# Autodesk Inventor assembly: gripperReference
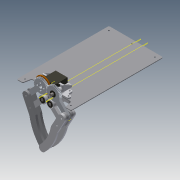
[picture p0: Inventor's stored thumbnail of the model, 180x180]
Saved by Autodesk Inventor 2018 (Build 220112000, 112)
## iProperties
Created: 2020-01-19
Part Number: gripperReference
Document SubType Name: Assembly
Designer: anirudh
Author: anirudh
## Documents named in this file (15)
- D:\Silicon Sharks\2019-2020\Gripper\gripperReference.iam
- D:\Silicon Sharks\2019-2020\Gripper\gripperServo.ipt
- D:\Silicon Sharks\2019-2020\Gripper\REV-41-1363.ipt
- D:\Silicon Sharks\2019-2020\Gripper\gripperPart1.ipt
- D:\Silicon Sharks\2019-2020\prototype3\bottomMountingPlate.ipt
- D:\Silicon Sharks\2019-2020\Gripper\gripperPart2.ipt
- D:\Silicon Sharks\2019-2020\Gripper\am-3377 6x12x4 Flanged Bearing.ipt
- D:\Silicon Sharks\2019-2020\Gripper\gripperPart3.ipt
- D:\Silicon Sharks\2019-2020\Gripper\gripperPart4.ipt
- D:\Silicon Sharks\2019-2020\Gripper\6mm-1inAxle.ipt
- D:\Silicon Sharks\2019-2020\Gripper\gripperPart5.ipt
- D:\Silicon Sharks\2019-2020\Gripper\spacer.ipt
- D:\Silicon Sharks\2019-2020\Gripper\servoMount.ipt
- D:\Silicon Sharks\2019-2020\Gripper\servoMount2.ipt
- D:\Silicon Sharks\2019-2020\Gripper\axleMount.ipt
## Components (26 placed, 14 different names)
1. gripperServo:1 — Mate:1, Mate:2, Mate:6, Flush:1, Flush:4, Mate:62, Mate:63, Mate:65, Mate:66
2. REV-41-1363:1 — Mate:1, Mate:2, Mate:3, Mate:4, Mate:5
3. gripperPart1:1 — Mate:3, Mate:4, Mate:5, Flush:7, Mate:18, Flush:10, Mate:34, Mate:35, Mate:38
4. bottomMountingPlate:1 — Mate:6, Flush:1, Flush:4, Flush:6, Mate:11, Flush:8, Mate:20, Mate:21, Flush:9, Mate:61, Mate:64, Flush:14
5. gripperPart2:1 — Flush:7, Mate:11, Mate:13, Mate:14, Mate:15, Mate:16, Mate:17, Mate:19, Flush:11, Mate:56, Mate:58, Mate:60
6. am-3377 6x12x4 Flanged Bearing:1 — Mate:14, Mate:15, Mate:68
7. am-3377 6x12x4 Flanged Bearing:2 — Mate:16, Mate:17, Mate:67
8. gripperPart3:1 — Mate:20, Mate:21, Flush:9, Mate:22, Mate:31, Flush:12, Mate:32, Flush:13, Mate:33
9. gripperPart4:1 — Flush:10, Mate:22, Mate:23, Mate:24, Mate:25, Mate:26, Mate:36, Mate:37, Mate:39
10. gripperPart4:2 — Mate:27, Mate:28, Mate:29, Mate:30, Flush:11, Mate:40, Mate:41, Mate:46, Mate:47
11. am-3377 6x12x4 Flanged Bearing:3 — Mate:25, Mate:26
12. am-3377 6x12x4 Flanged Bearing:4 — Mate:29, Mate:30, Mate:31
13. am-3377 6x12x4 Flanged Bearing:5 — Mate:27, Mate:28
14. am-3377 6x12x4 Flanged Bearing:6 — Mate:23, Mate:24
15. 6mm-1inAxle:1 — Flush:13, Mate:33
16. 6mm-1inAxle:2 — Flush:12, Mate:32
17. gripperPart5:1 — Mate:34, Mate:35, Mate:36
18. gripperPart5:2 — Mate:37, Mate:38, Mate:39
19. spacer:1 — Mate:40, Mate:41, Mate:50, Mate:54, Mate:55, Mate:60
20. spacer:4 — Mate:46, Mate:47, Mate:53, Mate:57, Mate:59
21. gripperPart5:3 — Mate:53, Mate:57, Mate:58, Mate:59
22. gripperPart5:4 — Mate:50, Mate:54, Mate:55, Mate:56
23. servoMount:1 — Mate:61, Mate:62, Mate:63
24. servoMount2:1 — Mate:64, Mate:65, Mate:66
25. axleMount:1 — Mate:67, Flush:14, Flush:15
26. 6mm-1inAxle:3 — Flush:15, Mate:68
## Relationships (67: Mate 55, Flush 12)
- Mate:1: gripperServo:1 ↔ REV-41-1363:1
- Mate:2: gripperServo:1 ↔ REV-41-1363:1
- Mate:3: REV-41-1363:1 ↔ gripperPart1:1
- Mate:4: REV-41-1363:1 ↔ gripperPart1:1
- Mate:5: REV-41-1363:1 ↔ gripperPart1:1
- Mate:6: gripperServo:1 ↔ bottomMountingPlate:1
- Flush:1: gripperServo:1 ↔ bottomMountingPlate:1
- Flush:4: gripperServo:1 ↔ bottomMountingPlate:1
- Flush:6 (7.493 mm): bottomMountingPlate:1
- Flush:7: gripperPart1:1 ↔ gripperPart2:1
- Mate:11: bottomMountingPlate:1 ↔ gripperPart2:1
- Mate:13: gripperPart2:1
- Mate:14: gripperPart2:1 ↔ am-3377 6x12x4 Flanged Bearing:1
- Mate:15: gripperPart2:1 ↔ am-3377 6x12x4 Flanged Bearing:1
- Mate:16: gripperPart2:1 ↔ am-3377 6x12x4 Flanged Bearing:2
- Mate:17: gripperPart2:1 ↔ am-3377 6x12x4 Flanged Bearing:2
- Flush:8 (23.241 mm): bottomMountingPlate:1
- Mate:18: gripperPart1:1
- Mate:19: gripperPart2:1
- Mate:20: bottomMountingPlate:1 ↔ gripperPart3:1
- Mate:21: bottomMountingPlate:1 ↔ gripperPart3:1
- Flush:9: bottomMountingPlate:1 ↔ gripperPart3:1
- Flush:10: gripperPart1:1 ↔ gripperPart4:1
- Mate:22: gripperPart3:1 ↔ gripperPart4:1
- Mate:23: gripperPart4:1 ↔ am-3377 6x12x4 Flanged Bearing:6
- Mate:24: gripperPart4:1 ↔ am-3377 6x12x4 Flanged Bearing:6
- Mate:25: gripperPart4:1 ↔ am-3377 6x12x4 Flanged Bearing:3
- Mate:26: gripperPart4:1 ↔ am-3377 6x12x4 Flanged Bearing:3
- Mate:27: gripperPart4:2 ↔ am-3377 6x12x4 Flanged Bearing:5
- Mate:28: gripperPart4:2 ↔ am-3377 6x12x4 Flanged Bearing:5
- Mate:29: gripperPart4:2 ↔ am-3377 6x12x4 Flanged Bearing:4
- Mate:30: gripperPart4:2 ↔ am-3377 6x12x4 Flanged Bearing:4
- Flush:11: gripperPart2:1 ↔ gripperPart4:2
- Mate:31: gripperPart3:1 ↔ am-3377 6x12x4 Flanged Bearing:4
- Flush:12: gripperPart3:1 ↔ 6mm-1inAxle:2
- Mate:32: gripperPart3:1 ↔ 6mm-1inAxle:2
- Flush:13: gripperPart3:1 ↔ 6mm-1inAxle:1
- Mate:33: gripperPart3:1 ↔ 6mm-1inAxle:1
- Mate:34: gripperPart1:1 ↔ gripperPart5:1
- Mate:35: gripperPart1:1 ↔ gripperPart5:1
- Mate:36: gripperPart4:1 ↔ gripperPart5:1
- Mate:37: gripperPart4:1 ↔ gripperPart5:2
- Mate:38: gripperPart1:1 ↔ gripperPart5:2
- Mate:39: gripperPart4:1 ↔ gripperPart5:2
- Mate:40: gripperPart4:2 ↔ spacer:1
- Mate:41: gripperPart4:2 ↔ spacer:1
- Mate:46: gripperPart4:2 ↔ spacer:4
- Mate:47: gripperPart4:2 ↔ spacer:4
- Mate:50: spacer:1 ↔ gripperPart5:4
- Mate:53: spacer:4 ↔ gripperPart5:3
- Mate:54: spacer:1 ↔ gripperPart5:4
- Mate:55: spacer:1 ↔ gripperPart5:4
- Mate:56: gripperPart2:1 ↔ gripperPart5:4
- Mate:57: spacer:4 ↔ gripperPart5:3
- Mate:58: gripperPart2:1 ↔ gripperPart5:3
- Mate:59: spacer:4 ↔ gripperPart5:3
- Mate:60: gripperPart2:1 ↔ spacer:1
- Mate:61: bottomMountingPlate:1 ↔ servoMount:1
- Mate:62: gripperServo:1 ↔ servoMount:1
- Mate:63: gripperServo:1 ↔ servoMount:1
- Mate:64: bottomMountingPlate:1 ↔ servoMount2:1
- Mate:65: gripperServo:1 ↔ servoMount2:1
- Mate:66: gripperServo:1 ↔ servoMount2:1
- Mate:67: am-3377 6x12x4 Flanged Bearing:2 ↔ axleMount:1
- Flush:14: bottomMountingPlate:1 ↔ axleMount:1
- Flush:15: axleMount:1 ↔ 6mm-1inAxle:3
- Mate:68: am-3377 6x12x4 Flanged Bearing:1 ↔ 6mm-1inAxle:3
